# Autodesk Inventor assembly: gusset
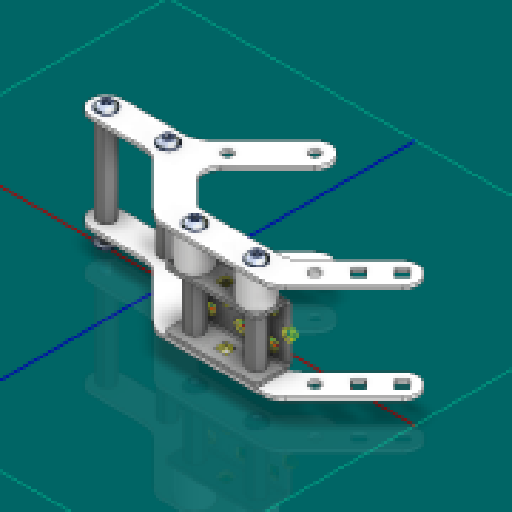
[picture p0: Inventor's stored thumbnail of the model, 512x512]
Saved by Autodesk Inventor 2025 (Build 290162000, 162)
## iProperties
Created: 2024-08-17
Part Number: gusset
Document SubType Name: Assembly
Designer: averey
Author: averey
## Documents named in this file (12)
- C:\Users\avere\vex_robotics_high_stakes\hardware\cad\ATLAS\chassis\drive_pod\gusset.iam
- C:\Users\avere\vex_robotics_high_stakes\hardware\cad\ATLAS\chassis\drive_pod\custom_parts\join_gusset.ipt
- C:\Users\avere\vex_robotics_high_stakes\hardware\cad\VEX-CAD-Inventor\Motion\Spacers\Spacer Nylon .500 OD\NSpacer White .500 OD x .500.ipt
- C:\Users\avere\vex_robotics_high_stakes\hardware\cad\VEX-CAD-Inventor\Motion\Spacers\Spacer Nylon .500 OD.ipt
- C:\Users\avere\vex_robotics_high_stakes\hardware\cad\VEX-CAD-Inventor\Structure\C Channel\Aluminum 1x2x1\Alu C 1x2x1x3.ipt
- C:\Users\avere\vex_robotics_high_stakes\hardware\cad\VEX-CAD-Inventor\Structure\Standoff\Standoff .875.ipt
- C:\Users\avere\vex_robotics_high_stakes\hardware\cad\VEX-CAD-Inventor\Structure\Standoff.ipt
- C:\Users\avere\vex_robotics_high_stakes\hardware\cad\VEX-CAD-Inventor\Structure\Hardware\Screw Steel - Star\SScrew Star Smooth .750.ipt
- C:\Users\avere\vex_robotics_high_stakes\hardware\cad\VEX-CAD-Inventor\Structure\Hardware\Screw Steel - Star.ipt
- C:\Users\avere\vex_robotics_high_stakes\hardware\cad\VEX-CAD-Inventor\Structure\Hardware\Screw Shoulder Robosource\SScrew Shoulder Smooth .375 x .12.ipt
- C:\Users\avere\vex_robotics_high_stakes\hardware\cad\VEX-CAD-Inventor\Structure\Hardware\Screw Shoulder Robosource.ipt
- C:\Users\avere\vex_robotics_high_stakes\hardware\cad\VEX-CAD-Inventor\Structure\Hardware\Screw Steel - Star\SScrew Star Smooth .290.ipt
## Components (15 placed, 7 different names)
1. join_gusset:1 — Insert:1, Mate:1, Insert:15, Insert:17
2. join_gusset:2 — Insert:1, Mate:1, Insert:5, Insert:7, Insert:13, Insert:14, Insert:31, Insert:32, Insert:33, Insert:34
3. NSpacer White .500 OD x .500:4 — Insert:5, Insert:8
4. NSpacer White .500 OD x .500:5 — Insert:7, Mate:2
5. Alu C 1x2x1x3:1 — Insert:8, Mate:2, Insert:9, Insert:10
6. Standoff .875:1 — Insert:9
7. Standoff .875:2 — Insert:10
8. SScrew Star Smooth .750:1 — Insert:14
9. SScrew Star Smooth .750:2 — Insert:13
10. SScrew Shoulder Smooth .375 x .12:1 — Insert:15
11. SScrew Shoulder Smooth .375 x .12:2 — Insert:17
12. SScrew Star Smooth .290:9 — Insert:31
13. SScrew Star Smooth .290:10 — Insert:32
14. NSpacer White .500 OD x .500:6 — Insert:33
15. NSpacer White .500 OD x .500:7 — Insert:34
## Relationships (16: Insert 14, Mate 2)
- Insert:1 (38.1 mm): join_gusset:1 ↔ join_gusset:2
- Mate:1: join_gusset:1 ↔ join_gusset:2
- Insert:5: join_gusset:2 ↔ NSpacer White .500 OD x .500:4
- Insert:7: join_gusset:2 ↔ NSpacer White .500 OD x .500:5
- Insert:8: NSpacer White .500 OD x .500:4 ↔ Alu C 1x2x1x3:1
- Mate:2: NSpacer White .500 OD x .500:5 ↔ Alu C 1x2x1x3:1
- Insert:9: Alu C 1x2x1x3:1 ↔ Standoff .875:1
- Insert:10: Alu C 1x2x1x3:1 ↔ Standoff .875:2
- Insert:13: join_gusset:2 ↔ SScrew Star Smooth .750:2
- Insert:14: join_gusset:2 ↔ SScrew Star Smooth .750:1
- Insert:15: join_gusset:1 ↔ SScrew Shoulder Smooth .375 x .12:1
- Insert:17: join_gusset:1 ↔ SScrew Shoulder Smooth .375 x .12:2
- Insert:31: join_gusset:2 ↔ SScrew Star Smooth .290:9
- Insert:32: join_gusset:2 ↔ SScrew Star Smooth .290:10
- Insert:33: join_gusset:2 ↔ NSpacer White .500 OD x .500:6
- Insert:34: join_gusset:2 ↔ NSpacer White .500 OD x .500:7
